# Autodesk Inventor assembly: XY Joint Right
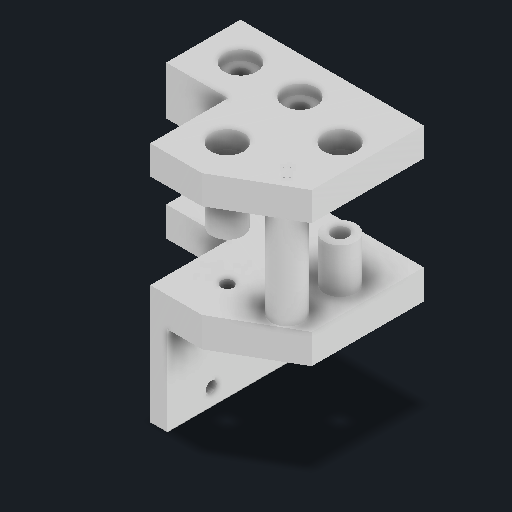
[picture p0: Inventor's stored thumbnail of the model, 512x512]
Saved by Autodesk Inventor 2025.1 (Build 291241020, 241B)
## iProperties
Created: 2025-04-19
Part Number: XY Joint Right
Document SubType Name: Assembly
Designer: Joshua Eah
Author: Joshua Eah
## Documents named in this file (5)
- C:\Users\Joshua Eah\Documents\Voron 0.2\CAD\Machined Parts\XY Joints\XY Joint Right\XY Joint Right.iam
- C:\Users\Joshua Eah\Documents\Voron 0.2\CAD\Machined Parts\XY Joints\XY Joint Right\XY Joint Right Lower.ipt
- C:\Users\Joshua Eah\Documents\Voron 0.2\CAD\Machined Parts\XY Joints\XY Joint Right\XY Joint Right Upper.ipt
- C:\Users\Joshua Eah\Documents\Voron 0.2\CAD\Machined Parts\XY Joints\XY Joint Support\XY Joint Support.ipt
- C:\Users\Joshua Eah\Documents\Voron 0.2\CAD\Machined Parts\Spacers\Spacer.ipt
## Components (5 placed, 4 different names)
1. XY Joint Right Lower:1 — Rigid:1, Mate:2
2. XY Joint Right Upper:1 — Rotational:1, Mate:1
3. XY Joint Support:1 — Rigid:1, Rotational:1
4. Spacer:1 — Mate:1
5. Spacer:2 — Mate:2
## Relationships (4: Mate 2, WeldJoint 1, RevoluteJoint 1)
- Rigid:1 [WeldJoint]: XY Joint Right Lower:1 ↔ XY Joint Support:1
- Rotational:1 [RevoluteJoint]: XY Joint Right Upper:1 ↔ XY Joint Support:1
- Mate:1: XY Joint Right Upper:1 ↔ Spacer:1
- Mate:2: XY Joint Right Lower:1 ↔ Spacer:2
